# Autodesk Inventor assembly: 300138-FR-001
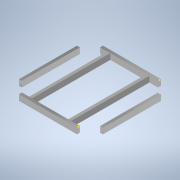
[picture p0: Inventor's stored thumbnail of the model, 180x180]
Saved by Autodesk Inventor 2022.2 (Build 262287000, 287)
## iProperties
_FrameDoc: Frame Assembly
_Version: 25.0.0
Created: 2022-09-15
Part Number: 300138-FR-001
Document SubType Name: Assembly
Designer: robotics
Mass: 3103.7 g
Surface Area: 9827.93 cm^2
Volume: 1578.17 cm^3
Density: 1.96664 g/cm^3
Author: robotics
## Documents named in this file (8)
- C:\$WorkingFolder\Projects\2022\Offseason\Swerve Drive\300138\Frame\300138-FR-001.iam
- C:\$WorkingFolder\Projects\2022\Offseason\Swerve Drive\300138\Frame\300138 Skeleton-0001.ipt
- C:\$WorkingFolder\Projects\2022\Offseason\Swerve Drive\300138\Frame\300138-FM-0001.ipt
- C:\$WorkingFolder\Projects\2022\Offseason\Swerve Drive\300138\Frame\300138-FM-0002.ipt
- C:\$WorkingFolder\Projects\2022\Offseason\Swerve Drive\300138\Frame\300138-FM-0003.ipt
- C:\$WorkingFolder\Projects\2022\Offseason\Swerve Drive\300138\Frame\300138-FM-0004.ipt
- C:\$WorkingFolder\Projects\2022\Offseason\Swerve Drive\200522.ipt
- C:\$WorkingFolder\Projects\2022\Offseason\Swerve Drive\200520.ipt
## Components (11 placed, 7 different names)
1. 300138 Skeleton-0001:1
2. 300138-FM-0001:1 — Mate:9, Flush:5, Mate:10, Flush:6
3. 300138-FM-0002:1
4. 300138-FM-0003:1 — Flush:8
5. 300138-FM-0004:1 — Flush:7
6. 200522:1 — Flush:1, Mate:1, Mate:2, Mate:9
7. 200522:2 — Flush:3, Mate:5, Mate:6
8. 200522:3 — Flush:4, Mate:7, Mate:8, Mate:10
9. 200522:4 — Flush:2, Mate:3, Mate:4
10. 200520:1 — Flush:1, Mate:1, Mate:2, Flush:2, Mate:3, Mate:4, Flush:5, Flush:7
11. 200520:2 — Flush:3, Mate:5, Mate:6, Flush:4, Mate:7, Mate:8, Flush:6, Flush:8
## Relationships (18: Mate 10, Flush 8)
- Flush:1: 200522:1 ↔ 200520:1
- Mate:1: 200522:1 ↔ 200520:1
- Mate:2: 200522:1 ↔ 200520:1
- Flush:2: 200522:4 ↔ 200520:1
- Mate:3: 200522:4 ↔ 200520:1
- Mate:4: 200522:4 ↔ 200520:1
- Flush:3: 200522:2 ↔ 200520:2
- Mate:5: 200522:2 ↔ 200520:2
- Mate:6: 200522:2 ↔ 200520:2
- Flush:4: 200522:3 ↔ 200520:2
- Mate:7: 200522:3 ↔ 200520:2
- Mate:8: 200522:3 ↔ 200520:2
- Mate:9: 300138-FM-0001:1 ↔ 200522:1
- Flush:5: 300138-FM-0001:1 ↔ 200520:1
- Mate:10: 300138-FM-0001:1 ↔ 200522:3
- Flush:6: 300138-FM-0001:1 ↔ 200520:2
- Flush:7 (190.5 mm): 300138-FM-0004:1 ↔ 200520:1
- Flush:8 (-190.5 mm): 300138-FM-0003:1 ↔ 200520:2
